# Autodesk Inventor assembly: FE-00040-01_ASM_8_ASM
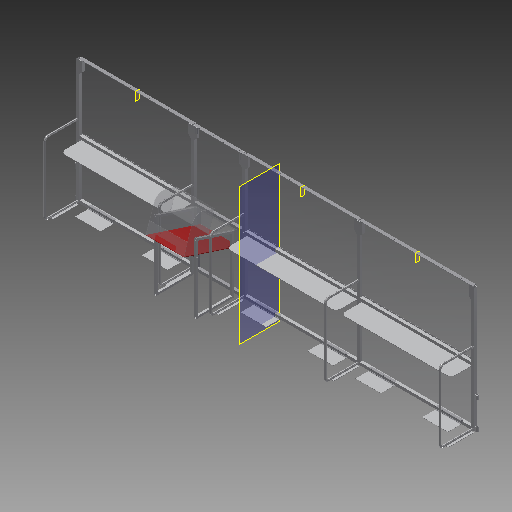
[picture p0: Inventor's stored thumbnail of the model, 512x512]
Saved by Autodesk Inventor 2017 (Build 210142000, 142)
## iProperties
Created: 2016-12-16
Part Number: FE-00040-01_ASM_8_ASM
Document SubType Name: Assembly
Designer: PhillipD
Author: PhillipD
Revision Number: 1LAST_VERSION
## Documents named in this file (8)
- C:\Users\jeff1\OneDrive\Documents\1504\217-2000-STEP\Parts\FE-00040-01_ASM_8_ASM.iam
- C:\Users\jeff1\OneDrive\Documents\1504\217-2000-STEP\Parts\FE-00002-L_ASM_2_ASM.iam
- C:\Users\jeff1\OneDrive\Documents\1504\217-2000-STEP\Parts\FE-00004_ASM_2_ASM.iam
- C:\Users\jeff1\OneDrive\Documents\1504\217-2000-STEP\Parts\FE-00001_ASM_3_ASM.iam
- C:\Users\jeff1\OneDrive\Documents\1504\217-2000-STEP\Parts\FE-00002-R_ASM_3_ASM.iam
- C:\Users\jeff1\OneDrive\Documents\1504\217-2000-STEP\Parts\FE-00007_ASM_2_ASM.iam
- C:\Users\jeff1\OneDrive\Documents\1504\217-2000-STEP\Parts\FE-00012_2.ipt
- C:\Users\jeff1\OneDrive\Documents\1504\217-2000-STEP\Parts\GE-17307_ASM_36_ASM_RED.iam
## Components (15 placed, 15 different names)
1. FE-00002-L_ASM_2_ASM_807 [sub-assembly] — Symmetry:1
2. FE-00004_ASM_2_ASM_839 [sub-assembly]
3. FE-00001_ASM_3_ASM_847 [sub-assembly]
4. GE-17307_ASM_36_ASM_873 [sub-assembly]
5. FE-00001_ASM_3_ASM_874 [sub-assembly]
6. FE-00004_ASM_2_ASM_875 [sub-assembly]
7. FE-00001_ASM_3_ASM_876 [sub-assembly]
8. FE-00004_ASM_2_ASM_877 [sub-assembly]
9. FE-00002-R_ASM_3_ASM_886 [sub-assembly] — Symmetry:1
10. FE-00007_ASM_2_ASM_891 [sub-assembly]
11. FE-00007_ASM_2_ASM_892 [sub-assembly]
12. FE-00007_ASM_2_ASM_893 [sub-assembly]
13. FE-00012_2_894
14. FE-00012_2_895
15. FE-00012_2_896
## Relationships (1: Symmetry 1)
- Symmetry:1: FE-00002-L_ASM_2_ASM_807 ↔ FE-00002-R_ASM_3_ASM_886
